# Autodesk Inventor assembly: rev1
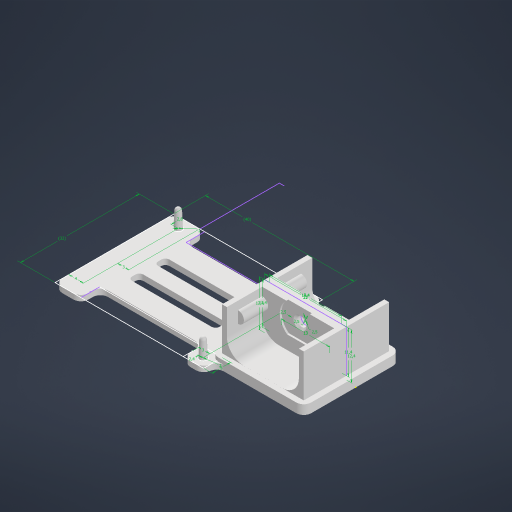
[picture p0: Inventor's stored thumbnail of the model, 512x512]
Saved by Autodesk Inventor 2024 (Build 280153000, 153)
## iProperties
Created: 2023-10-23
Part Number: rev1
Document SubType Name: Assembly
Designer: 21guslof
Author: 21guslof
## Documents named in this file (3)
- C:\Users\Gurra\Documents\GitRepos\MDU-SamarbetanderobotarDVA138\Projekt\CAD\NewProduction\rev1.iam
- C:\Users\Gurra\Documents\GitRepos\MDU-SamarbetanderobotarDVA138\Projekt\CAD\NewProduction\MotorHolder.ipt
- C:\Users\Gurra\Documents\GitRepos\MDU-SamarbetanderobotarDVA138\Projekt\CAD\NewProduction\Baseplate.ipt
## Components (3 placed, 2 different names)
1. MotorHolder:1 — Mate:1, Flush:1, Flush:2
2. Baseplate:1 — Mate:2, Mate:3, Mate:4
3. MotorHolder:2 — Mate:1, Flush:1, Flush:2, Mate:2, Mate:3, Mate:4
## Relationships (6: Mate 4, Flush 2)
- Mate:1: MotorHolder:1 ↔ MotorHolder:2
- Flush:1: MotorHolder:1 ↔ MotorHolder:2
- Flush:2: MotorHolder:1 ↔ MotorHolder:2
- Mate:2: Baseplate:1 ↔ MotorHolder:2
- Mate:3: Baseplate:1 ↔ MotorHolder:2
- Mate:4: Baseplate:1 ↔ MotorHolder:2
